# Autodesk Inventor assembly: Ensamblado
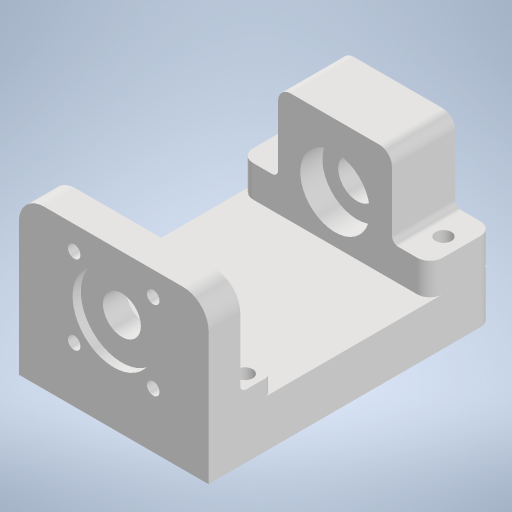
[picture p0: Inventor's stored thumbnail of the model, 512x512]
Saved by Autodesk Inventor 2023 (Build 270158000, 158)
## iProperties
Created: 2023-03-15
Part Number: Ensamblado
Document SubType Name: Assembly
Designer: Francisco
Author: Francisco
## Documents named in this file (4)
- D:\Universidad\Otros\Padrino tecnológico\Adaptador Soportes motor-rueda\Ensamblado.iam
- D:\Universidad\Otros\Padrino tecnológico\Adaptador Soportes motor-rueda\Adaptador_soporte_motor-rueda.ipt
- D:\Universidad\Otros\Padrino tecnológico\Adaptador Soportes motor-rueda\SRE_2023_50_Soporte_rueda_aluminio.ipt
- D:\Universidad\Otros\Padrino tecnológico\Adaptador Soportes motor-rueda\SRE_2023_49_Soporte_motor_aluminio.ipt
## Components (3 placed, 3 different names)
1. Adaptador_soporte_motor-rueda:1 — Mate:1, Flush:1, Flush:2, Mate:2, Flush:3, Flush:4
2. SRE_2023_50_Soporte_rueda_aluminio:1 — Mate:1, Flush:1, Flush:2
3. SRE_2023_49_Soporte_motor_aluminio:1 — Mate:2, Flush:3, Flush:4
## Relationships (6: Flush 4, Mate 2)
- Mate:1: Adaptador_soporte_motor-rueda:1 ↔ SRE_2023_50_Soporte_rueda_aluminio:1
- Flush:1: Adaptador_soporte_motor-rueda:1 ↔ SRE_2023_50_Soporte_rueda_aluminio:1
- Flush:2: Adaptador_soporte_motor-rueda:1 ↔ SRE_2023_50_Soporte_rueda_aluminio:1
- Mate:2: Adaptador_soporte_motor-rueda:1 ↔ SRE_2023_49_Soporte_motor_aluminio:1
- Flush:3: Adaptador_soporte_motor-rueda:1 ↔ SRE_2023_49_Soporte_motor_aluminio:1
- Flush:4: Adaptador_soporte_motor-rueda:1 ↔ SRE_2023_49_Soporte_motor_aluminio:1
